# Autodesk Inventor assembly: Extrusora ensamblaje 2
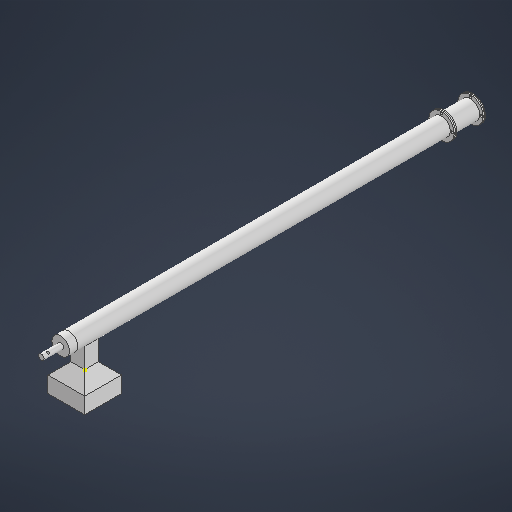
[picture p0: Inventor's stored thumbnail of the model, 512x512]
Saved by Autodesk Inventor 2026.1 (Build 301233020, 233B)
## iProperties
Created: 2025-12-03
Part Number: Extrusora ensamblaje 2
Document SubType Name: Assembly
Designer: benja
Author: benja
## Documents named in this file (9)
- C:\Users\benja\OneDrive\Escritorio\extrusora\Extrusora ensamblaje 2.iam
- C:\Users\benja\OneDrive\Escritorio\extrusora\alimentaciion tornillo .ipt
- C:\Users\benja\OneDrive\Escritorio\extrusora\compresion tornillo.ipt
- C:\Users\benja\OneDrive\Escritorio\extrusora\dosificacion tornillo.ipt
- C:\Users\benja\OneDrive\Escritorio\extrusora\tolva completa.iam
- C:\Users\benja\OneDrive\Escritorio\extrusora\tapa seccion alimentacion.ipt
- C:\Users\benja\OneDrive\Escritorio\extrusora\6201-c-2z.ipt
- C:\Users\benja\OneDrive\Escritorio\extrusora\cabezal extrusora.ipt
- C:\Users\benja\OneDrive\Escritorio\extrusora\placa para pellet.ipt
## Components (8 placed, 8 different names)
1. alimentaciion tornillo :1 — Coincidencia:1, Coincidencia:2, Coincidencia:3, Rotación:2, Coincidencia:7, Rotación:3, Coincidencia:9, Nivelación:1
2. compresion tornillo:1 — Coincidencia:1, Coincidencia:2, Coincidencia:3, Coincidencia:4, Coincidencia:5, Coincidencia:6, Rotación:1, Rotación:2
3. dosificacion tornillo:1 — Coincidencia:4, Coincidencia:5, Coincidencia:6, Rotación:1, Rotación:3
4. tolva completa:1 [sub-assembly] — Coincidencia:7, Nivelación:1, Coincidencia:10, Coincidencia:11, Coincidencia:14, Coincidencia:15
5. tapa seccion alimentacion:1 — Coincidencia:8, Tangente:1, Coincidencia:9, Coincidencia:10
6. 6201-c-2z:1 — Coincidencia:8, Tangente:1
7. cabezal extrusora:1 — Coincidencia:11, Coincidencia:13, Coincidencia:14, Coincidencia:15, Coincidencia:16, Coincidencia:17
8. placa para pellet:1 — Coincidencia:13, Coincidencia:16, Coincidencia:17
## Relationships (21: Mate 16, RelateRotation 3, Tangent 1, Flush 1)
- Coincidencia:1 [Mate]: alimentaciion tornillo :1 ↔ compresion tornillo:1
- Coincidencia:2 [Mate]: alimentaciion tornillo :1 ↔ compresion tornillo:1
- Coincidencia:3 [Mate]: alimentaciion tornillo :1 ↔ compresion tornillo:1
- Coincidencia:4 [Mate]: compresion tornillo:1 ↔ dosificacion tornillo:1
- Coincidencia:5 [Mate]: compresion tornillo:1 ↔ dosificacion tornillo:1
- Coincidencia:6 [Mate]: compresion tornillo:1 ↔ dosificacion tornillo:1
- Rotación:1 [RelateRotation] (1 ul): compresion tornillo:1 ↔ dosificacion tornillo:1
- Rotación:2 [RelateRotation] (1.356 ul): alimentaciion tornillo :1 ↔ compresion tornillo:1
- Coincidencia:7 [Mate]: alimentaciion tornillo :1 ↔ tolva completa:1
- Rotación:3 [RelateRotation] (0.914 ul): alimentaciion tornillo :1 ↔ dosificacion tornillo:1
- Coincidencia:8 [Mate]: tapa seccion alimentacion:1 ↔ 6201-c-2z:1
- Tangente:1: tapa seccion alimentacion:1 ↔ 6201-c-2z:1
- Coincidencia:9 [Mate]: alimentaciion tornillo :1 ↔ tapa seccion alimentacion:1
- Nivelación:1 [Flush]: alimentaciion tornillo :1 ↔ tolva completa:1
- Coincidencia:10 [Mate]: tolva completa:1 ↔ tapa seccion alimentacion:1
- Coincidencia:11 [Mate]: tolva completa:1 ↔ cabezal extrusora:1
- Coincidencia:13 [Mate]: cabezal extrusora:1 ↔ placa para pellet:1
- Coincidencia:14 [Mate]: tolva completa:1 ↔ cabezal extrusora:1
- Coincidencia:15 [Mate]: tolva completa:1 ↔ cabezal extrusora:1
- Coincidencia:16 [Mate]: cabezal extrusora:1 ↔ placa para pellet:1
- Coincidencia:17 [Mate]: cabezal extrusora:1 ↔ placa para pellet:1
